# Autodesk Inventor assembly: Motor
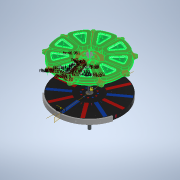
[picture p0: Inventor's stored thumbnail of the model, 180x180]
Saved by Autodesk Inventor 2022.2 (Build 262287000, 287)
## iProperties
Created: 2022-07-30
Part Number: Motor
Document SubType Name: Assembly
Designer: ABL
Author: ABL
## Documents named in this file (7)
- C:\GitHubRepos\PHYS-12-Website\content\portfolio\Final Project\CAD\Motor.iam
- C:\GitHubRepos\PHYS-12-Website\content\portfolio\Final Project\CAD\Stator.iam
- C:\GitHubRepos\PHYS-12-Website\content\portfolio\Final Project\CAD\Rotor.iam
- C:\GitHubRepos\PHYS-12-Website\content\portfolio\Final Project\CAD\FlangeBearing.ipt
- C:\GitHubRepos\PHYS-12-Website\content\portfolio\Final Project\CAD\Shaft.ipt
- C:\GitHubRepos\PHYS-12-Website\content\portfolio\Final Project\CAD\FlangeCoupling.ipt
- C:\GitHubRepos\PHYS-12-Website\content\portfolio\Final Project\CAD\MotorGlobalParameters.xlsx
## Components (6 placed, 5 different names)
1. Stator:1 [sub-assembly] — Flush:1, Mate:6
2. Rotor:1 [sub-assembly] — Mate:1, Mate:3, Cylindrical:2, Mate:4, Flush:1
3. FlangeBearing:1 — Mate:1, Mate:7
4. FlangeBearing:2 — Mate:3, Mate:4
5. Shaft:1 — Cylindrical:2, Mate:5, Mate:7
6. FlangeCoupling:1 — Mate:5, Mate:6
## Relationships (8: Mate 6, CylindricalJoint 1, Flush 1)
- Mate:1: Rotor:1 ↔ FlangeBearing:1
- Mate:3: Rotor:1 ↔ FlangeBearing:2
- Cylindrical:2: Rotor:1 ↔ Shaft:1
- Mate:4: Rotor:1 ↔ FlangeBearing:2
- Flush:1: Stator:1 ↔ Rotor:1
- Mate:5: Shaft:1 ↔ FlangeCoupling:1
- Mate:6: Stator:1 ↔ FlangeCoupling:1
- Mate:7: FlangeBearing:1 ↔ Shaft:1
## Named parameters: gap = 0.1 mm, airgap = 0.4 mm, wallgap = 2 mm, driveMagnet_length = 60 mm, driveMagnet_width = 10 mm, driveMagnet_height = 5 mm, driveMagnet_numStacked = 2, halbachMagnet_length = 60 mm, halbachMagnet_width = 10 mm, halbachMagnet_height = 3 mm, halbachMagnet_numStacked = 2, rotorBandBolt_diameter = 2 mm, rotorBandBolt_headDiameter = 3.98 mm, rotorBandBolt_headHeight = 2 mm, rotorBandBolt_shaftLength = 20 mm, rotorBandHexNut_sideToSide = 4 mm, rotorBandHexNut_height = 1.2 mm, rotorBandSquareNut_sideLength = 4 mm, rotorBandSquareNut_height = 1.2 mm, sensorMagnet_diameter = 5 mm, sensorMagnet_height = 2.66667 mm, numMagnetSets = 12, numElectromagnets = 9, driveMagnet_centerSpacingRadius = 38.96113 mm, rotorRadius = 101.16113 mm, rotorThickness = 14.1 mm, rotor_mountingLipHeight = 8 mm, shaftDiameter = 8 mm, flangeBearing_innerDiameter = 8 mm, flangeBearing_outerDiameter = 16 mm, flangeBearing_flangeDiameter = 18 mm, flangeBearing_height = 5 mm, flangeBearing_flangeHeight = 1 mm, statorThickness = 16 mm, rotorBandThickness = 4.1 mm, shaftLength = 200 mm, flangeCoupling_collarOuterDiameter = 16 mm, flangeCoupling_flangeHoleEdgeToEdge = 2.05 mm, flangeCoupling_innerDiameter = 8 mm, flangeCoupling_flangeHoleDiameter = 3.9 mm, flangeCoupling_flangeHeight = 3.1 mm, flangeCoupling_collarHeight = 10 mm, flangeCoupling_flangeDiameter = 32 mm, flangeCoupling_height = 13.1 mm, flangeCoupling_mountHoleDiameter = 3.9 mm, flangeCoupling_mountHoleEdgeToEdge = 2.05 mm, statorRadius = 99.16113 mm, coilThickness = 12 mm, statorMountBolt_diameter = 4 mm, statorMountBolt_headDiameter = 7 mm, statorMountBolt_headHeight = 4 mm, statorMountBolt_shaftLength = 17.1 mm, statorMountHexNut_height = 4 mm, statorMountHexNut_sideToSide = 8 mm, sensorMagnet_ringRadius = 23.48057 mm, coil_percentCoverage = 0.6, statorSpokeDegrees = 4 deg, coil_bulge = 3 mm, coil_cornerRadius = 10 mm, coil_width = 10 mm, statorCoilBolt_shaftLength = 12 mm, statorCoilHexNut_height = 1.2 mm, statorCoilBolt_headHeight = 2 mm, statorCoilBolt_diameter = 2 mm, statorCoilBolt_headDiameter = 3.98 mm, statorCoilHexNut_sideToSide = 4 mm, magnetWire_gauge = 20, magnetWire_outerDiameter = 0.8128 mm, printingLayerHeight = 0.2 mm, circuitBoard_height = 1.6 mm, hallEffectSensor_width = 1.6 mm, hallEffectSensor_length = 3 mm, hallEffectSensor_height = 1.1 mm, hallEffectSensor_pinLength = 0.6 mm, circuitboardMountHexNut_height = 1.2 mm, circuitboardMountHexNut_sideToSide = 4 mm, circuitboardMountBolt_headHeight = 2 mm, circuitboardMountBolt_shaftLength = 12 mm, circuitboardMountBolt_diameter = 2 mm, circuitboardMountBolt_headDiameter = 3.98 mm, statorShellBolt_headDiameter = 5.68 mm, statorShellHexNut_height = 2.3 mm, statorShellBolt_shaftLength = 12.6 mm, statorShellBolt_headHeight = 3 mm, statorShellHexNut_sideToSide = 5.3 mm, statorShellBolt_diameter = 3 mm, statorShellBolt_countersinkDepth = 3.4 mm
